# Autodesk Inventor assembly: Full Wheel Configuration
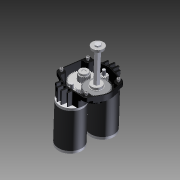
[picture p0: Inventor's stored thumbnail of the model, 180x180]
Saved by Autodesk Inventor 2015 (Build 190159000, 159)
## iProperties
Created: 2015-01-17
Part Number: Full Wheel Configuration
Document SubType Name: Assembly
Designer: jhirshland1
Author: jhirshland1
## Documents named in this file (3)
- C:\Users\jhirshland1\Inventor\HWRobot2015\FRCKOP2015\AndyMark\Full Wheel Configuration.iam
- C:\Users\jhirshland1\Inventor\HWRobot2015\FRCKOP2015\Drive Base\Toughbox Mini L-Base.iam
- C:\Users\jhirshland1\Inventor\HWRobot2015\FRCKOP2015\Drive Base\FR8ZZ Hex Bearing.ipt
## Components (2 placed, 2 different names)
1. Toughbox Mini L-Base:1 [sub-assembly]
2. FR8ZZ Hex Bearing:1
## Relationships (2: Mate 2)
- [Mate]: Toughbox Mini L-Base:1 ↔ FR8ZZ Hex Bearing:1
- [Mate]: Toughbox Mini L-Base:1 ↔ FR8ZZ Hex Bearing:1
